# Autodesk Inventor assembly: ENSAMBLADO
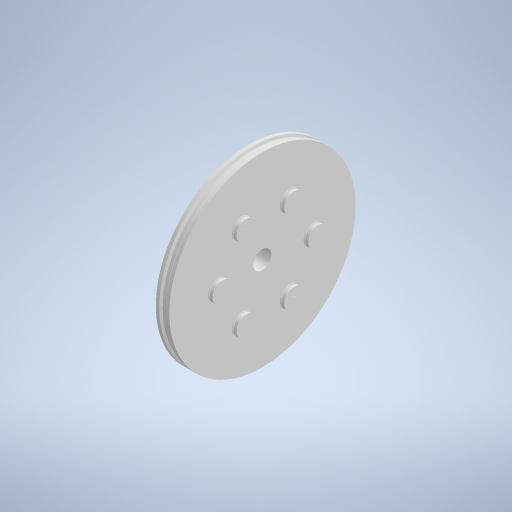
[picture p0: Inventor's stored thumbnail of the model, 512x512]
Saved by Autodesk Inventor 2024 (Build 280153000, 153)
## iProperties
Created: 2024-03-31
Part Number: ENSAMBLADO
Document SubType Name: Assembly
Designer: benja
Author: benja
## Documents named in this file (6)
- C:\Users\benja\Downloads\ENSAMBLADO.iam
- C:\Users\benja\Downloads\POLEA.ipt
- C:\Users\benja\Downloads\ENGRANE.ipt
- C:\Users\benja\Downloads\EJE_CUÑEROS.ipt
- C:\Users\benja\Downloads\CUÑA.ipt
- C:\Users\benja\Downloads\Parte 4.ipt
## Components (31 placed, 5 different names)
1. POLEA:1 — Cylindrical:1, Flush:1
2. ENGRANE:1 — Cylindrical:2, Flush:2
3. EJE_CUÑEROS:1 — Cylindrical:1, Flush:1, Cylindrical:2, Flush:2, Planar:1, Mate:1, Mate:2, Planar:2, Mate:3, Mate:4, Rotational:1
4. CUÑA:1 — Planar:1, Mate:1, Mate:2
5. CUÑA:3 — Planar:2, Mate:3, Mate:4
6. Parte 4:1 — Rotational:1, Rotational:2, Rotational:3, Rotational:4, Rotational:5, Rotational:6, Flush:13
7. POLEA:2
8. ENGRANE:2
9. EJE_CUÑEROS:2 — Rotational:6
10. CUÑA:4
11. CUÑA:5
12. POLEA:3
13. ENGRANE:3
14. EJE_CUÑEROS:3 — Rotational:3
15. CUÑA:6
16. CUÑA:7
17. POLEA:4
18. ENGRANE:4
19. EJE_CUÑEROS:4 — Rotational:4
20. CUÑA:8
21. CUÑA:9
22. POLEA:5
23. ENGRANE:5
24. EJE_CUÑEROS:5 — Rotational:5, Flush:13
25. CUÑA:10
26. CUÑA:11
27. POLEA:6
28. ENGRANE:6
29. EJE_CUÑEROS:6 — Rotational:2
30. CUÑA:12
31. CUÑA:13
## Relationships (67: Mate 24, Flush 13, CylindricalJoint 12, PlanarJoint 12, RevoluteJoint 6)
- Cylindrical:1: POLEA:1 ↔ EJE_CUÑEROS:1
- Flush:1: POLEA:1 ↔ EJE_CUÑEROS:1
- Cylindrical:2: ENGRANE:1 ↔ EJE_CUÑEROS:1
- Flush:2 (5.08 mm): ENGRANE:1 ↔ EJE_CUÑEROS:1
- Planar:1: EJE_CUÑEROS:1 ↔ CUÑA:1
- Mate:1: EJE_CUÑEROS:1 ↔ CUÑA:1
- Mate:2: EJE_CUÑEROS:1 ↔ CUÑA:1
- Planar:2: EJE_CUÑEROS:1 ↔ CUÑA:3
- Mate:3: EJE_CUÑEROS:1 ↔ CUÑA:3
- Mate:4: EJE_CUÑEROS:1 ↔ CUÑA:3
- [CylindricalJoint]: POLEA:2 ↔ EJE_CUÑEROS:2
- [Flush]: POLEA:2 ↔ EJE_CUÑEROS:2
- [CylindricalJoint]: ENGRANE:2 ↔ EJE_CUÑEROS:2
- [Flush] (5.08 mm): ENGRANE:2 ↔ EJE_CUÑEROS:2
- [PlanarJoint]: EJE_CUÑEROS:2 ↔ CUÑA:4
- [Mate]: EJE_CUÑEROS:2 ↔ CUÑA:4
- [Mate]: EJE_CUÑEROS:2 ↔ CUÑA:4
- [PlanarJoint]: EJE_CUÑEROS:2 ↔ CUÑA:5
- [Mate]: EJE_CUÑEROS:2 ↔ CUÑA:5
- [Mate]: EJE_CUÑEROS:2 ↔ CUÑA:5
- [CylindricalJoint]: POLEA:3 ↔ EJE_CUÑEROS:3
- [Flush]: POLEA:3 ↔ EJE_CUÑEROS:3
- [CylindricalJoint]: ENGRANE:3 ↔ EJE_CUÑEROS:3
- [Flush] (5.08 mm): ENGRANE:3 ↔ EJE_CUÑEROS:3
- [PlanarJoint]: EJE_CUÑEROS:3 ↔ CUÑA:6
- [Mate]: EJE_CUÑEROS:3 ↔ CUÑA:6
- [Mate]: EJE_CUÑEROS:3 ↔ CUÑA:6
- [PlanarJoint]: EJE_CUÑEROS:3 ↔ CUÑA:7
- [Mate]: EJE_CUÑEROS:3 ↔ CUÑA:7
- [Mate]: EJE_CUÑEROS:3 ↔ CUÑA:7
- [CylindricalJoint]: POLEA:4 ↔ EJE_CUÑEROS:4
- [Flush]: POLEA:4 ↔ EJE_CUÑEROS:4
- [CylindricalJoint]: ENGRANE:4 ↔ EJE_CUÑEROS:4
- [Flush] (5.08 mm): ENGRANE:4 ↔ EJE_CUÑEROS:4
- [PlanarJoint]: EJE_CUÑEROS:4 ↔ CUÑA:8
- [Mate]: EJE_CUÑEROS:4 ↔ CUÑA:8
- [Mate]: EJE_CUÑEROS:4 ↔ CUÑA:8
- [PlanarJoint]: EJE_CUÑEROS:4 ↔ CUÑA:9
- [Mate]: EJE_CUÑEROS:4 ↔ CUÑA:9
- [Mate]: EJE_CUÑEROS:4 ↔ CUÑA:9
- [CylindricalJoint]: POLEA:5 ↔ EJE_CUÑEROS:5
- [Flush]: POLEA:5 ↔ EJE_CUÑEROS:5
- [CylindricalJoint]: ENGRANE:5 ↔ EJE_CUÑEROS:5
- [Flush] (5.08 mm): ENGRANE:5 ↔ EJE_CUÑEROS:5
- [PlanarJoint]: EJE_CUÑEROS:5 ↔ CUÑA:10
- [Mate]: EJE_CUÑEROS:5 ↔ CUÑA:10
- [Mate]: EJE_CUÑEROS:5 ↔ CUÑA:10
- [PlanarJoint]: EJE_CUÑEROS:5 ↔ CUÑA:11
- [Mate]: EJE_CUÑEROS:5 ↔ CUÑA:11
- [Mate]: EJE_CUÑEROS:5 ↔ CUÑA:11
- [CylindricalJoint]: POLEA:6 ↔ EJE_CUÑEROS:6
- [Flush]: POLEA:6 ↔ EJE_CUÑEROS:6
- [CylindricalJoint]: ENGRANE:6 ↔ EJE_CUÑEROS:6
- [Flush] (5.08 mm): ENGRANE:6 ↔ EJE_CUÑEROS:6
- [PlanarJoint]: EJE_CUÑEROS:6 ↔ CUÑA:12
- [Mate]: EJE_CUÑEROS:6 ↔ CUÑA:12
- [Mate]: EJE_CUÑEROS:6 ↔ CUÑA:12
- [PlanarJoint]: EJE_CUÑEROS:6 ↔ CUÑA:13
- [Mate]: EJE_CUÑEROS:6 ↔ CUÑA:13
- [Mate]: EJE_CUÑEROS:6 ↔ CUÑA:13
- Rotational:1 [RevoluteJoint] (-38.1 mm): EJE_CUÑEROS:1 ↔ Parte 4:1
- Rotational:2 [RevoluteJoint] (-38.1 mm): Parte 4:1 ↔ EJE_CUÑEROS:6
- Rotational:3 [RevoluteJoint] (-38.1 mm): Parte 4:1 ↔ EJE_CUÑEROS:3
- Rotational:4 [RevoluteJoint] (-38.1 mm): Parte 4:1 ↔ EJE_CUÑEROS:4
- Rotational:5 [RevoluteJoint] (-38.1 mm): Parte 4:1 ↔ EJE_CUÑEROS:5
- Rotational:6 [RevoluteJoint] (-38.1 mm): Parte 4:1 ↔ EJE_CUÑEROS:2
- Flush:13: Parte 4:1 ↔ EJE_CUÑEROS:5
## Named parameters: d14_d0 = -163.546337 deg, d15_d1 = -14.50197 mm, d16_d2 = 0 mm, d17_d3 = 163.546337 deg, d18_d4 = -9.42197 mm, d19_d5 = 5.08 mm, d20_d6 = 0 mm, d21_d7 = 0 mm, d22_d8 = 0 mm, d23_d11 = 0 mm, d24_d12 = 0 mm, d25_d13 = 0 mm, d26_d0 = -141.67635 deg, d27_d1 = -14.50197 mm, d28_d2 = 0 mm, d29_d3 = 141.67635 deg, d30_d4 = -9.42197 mm, d31_d5 = 5.08 mm, d32_d6 = 0 mm, d33_d7 = 0 mm, d34_d8 = 0 mm, d35_d11 = 0 mm, d36_d12 = 0 mm, d37_d13 = 0 mm, d38_d0 = -174.888954 deg, d39_d1 = -14.50197 mm, d40_d2 = 0 mm, d41_d3 = 174.888954 deg, d42_d4 = -9.42197 mm, d43_d5 = 5.08 mm, d44_d6 = 0 mm, d45_d7 = 0 mm, d46_d8 = 0 mm, d47_d11 = 0 mm, d48_d12 = 0 mm, d49_d13 = 0 mm, d50_d0 = 151.234745 deg, d51_d1 = -14.50197 mm, d52_d2 = 0 mm, d53_d3 = -151.234745 deg, d54_d4 = -9.42197 mm, d55_d5 = 5.08 mm, d56_d6 = 0 mm, d57_d7 = 0 mm, d58_d8 = 0 mm, d59_d11 = 0 mm, d60_d12 = 0 mm, d61_d13 = 0 mm, d62_d0 = 98.691657 deg, d63_d1 = -14.50197 mm, d64_d2 = 0 mm, d65_d3 = -98.691657 deg, d66_d4 = -9.42197 mm, d67_d5 = 5.08 mm, d68_d6 = 0 mm, d69_d7 = 0 mm, d70_d8 = 0 mm, d71_d11 = 0 mm, d72_d12 = 0 mm, d73_d13 = 0 mm
